# Autodesk Inventor assembly: Sledge
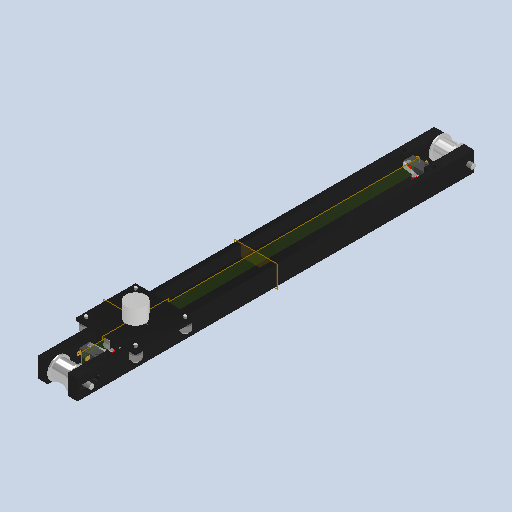
[picture p0: Inventor's stored thumbnail of the model, 512x512]
Saved by Autodesk Inventor 2025.1 (Build 291241020, 241B)
## iProperties
Created: 2024-11-07
Part Number: Sledge
Document SubType Name: Assembly
Designer: leon-
Author: leon-
## Documents named in this file (6)
- C:\Users\leon-\OneDrive\Dokumente\Education\Berkeley\Embedded_Systems\Project\CAD Model\Sledge.iam
- C:\Users\leon-\OneDrive\Dokumente\Education\Berkeley\Embedded_Systems\Project\CAD Model\Sledge_rail.ipt
- C:\Users\leon-\OneDrive\Dokumente\Education\Berkeley\Embedded_Systems\Project\CAD Model\Sledge_Assembly.iam
- C:\Users\leon-\OneDrive\Dokumente\Education\Berkeley\Embedded_Systems\Project\CAD Model\Available_Parts\MSW\MSW-13-17.iam
- MSW-13-17.iam
- C:\Users\leon-\OneDrive\Dokumente\Education\Berkeley\Embedded_Systems\Project\CAD Model\Bearing_Belt_Assembly.iam
## Components (6 placed, 4 different names)
1. Sledge_rail:1 — Tangent:1, Tangent:2, Tangent:3, Tangent:4, Tangent:5, Tangent:6, Mate:1, Mate:2, Mate:3, Mate:4, Mate:5, Mate:6, Mate:8, Tangent:7, Mate:9, Mate:10
2. Sledge_Assembly:1 [sub-assembly] — Tangent:1, Tangent:2, Tangent:3, Tangent:4, Tangent:5, Tangent:6
3. MSW-13-17:1 [sub-assembly] — Mate:1, Mate:2, Mate:3
4. MSW-13-17:2 [sub-assembly] — Mate:4, Mate:5, Mate:6
5. Bearing_Belt_Assembly:1 [sub-assembly] — Mate:8, Tangent:7
6. Bearing_Belt_Assembly:2 [sub-assembly] — Mate:9, Mate:10
## Relationships (16: Mate 9, Tangent 7)
- Tangent:1: Sledge_rail:1 ↔ Sledge_Assembly:1
- Tangent:2: Sledge_rail:1 ↔ Sledge_Assembly:1
- Tangent:3: Sledge_rail:1 ↔ Sledge_Assembly:1
- Tangent:4: Sledge_rail:1 ↔ Sledge_Assembly:1
- Tangent:5: Sledge_rail:1 ↔ Sledge_Assembly:1
- Tangent:6: Sledge_rail:1 ↔ Sledge_Assembly:1
- Mate:1: Sledge_rail:1 ↔ MSW-13-17:1
- Mate:2: Sledge_rail:1 ↔ MSW-13-17:1
- Mate:3: Sledge_rail:1 ↔ MSW-13-17:1
- Mate:4: Sledge_rail:1 ↔ MSW-13-17:2
- Mate:5: Sledge_rail:1 ↔ MSW-13-17:2
- Mate:6: Sledge_rail:1 ↔ MSW-13-17:2
- Mate:8: Sledge_rail:1 ↔ Bearing_Belt_Assembly:1
- Tangent:7: Sledge_rail:1 ↔ Bearing_Belt_Assembly:1
- Mate:9: Sledge_rail:1 ↔ Bearing_Belt_Assembly:2
- Mate:10: Sledge_rail:1 ↔ Bearing_Belt_Assembly:2
